# Autodesk Inventor assembly: 21.1846 LEVELING FOOT M10 WITH BORES
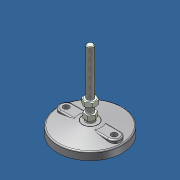
[picture p0: Inventor's stored thumbnail of the model, 180x180]
Saved by Autodesk Inventor 2016 (Build 200138000, 138)
## iProperties
Created: 2007-03-29
Part Number: 21.1846 LEVELING FOOT M10 WITH BORES
Document SubType Name: Assembly
Designer: Andy Moles
Author: Andy Moles
## Documents named in this file (5)
- C:\Users\myhome\Documents\Inventor\Printer\21.1846 LEVELING FOOT M10 WITH BORES.iam
- C:\Users\myhome\Documents\Inventor\Printer\LevelingFeet\ANTI-SKID PAD 100mm WITH BORES.ipt
- C:\Users\myhome\Documents\Inventor\Printer\LevelingFeet\PAD 100mm GRAY PLASTIC WITH BORES.IPT
- C:\Users\myhome\Documents\Inventor\Printer\LevelingFeet\21.1846 THREADED STUD 10mm.ipt
- C:\Users\myhome\Documents\Inventor\Printer\LevelingFeet\HEX NUT M10 DIN 934.ipt
## Components (4 placed, 4 different names)
1. ANTI-SKID PAD 100mm WITH BORES:1 — Insert:1, Mate:4
2. PAD 100mm GRAY PLASTIC WITH BORES:1 — Insert:1, Tangent:1, Mate:1, Mate:4
3. 21.1846 THREADED STUD 10mm:1 — Tangent:1, Mate:1, Mate:2
4. M10 HEX NUT DIN 934:1 — Mate:2
## Relationships (5: Mate 3, Insert 1, Tangent 1)
- Insert:1: ANTI-SKID PAD 100mm WITH BORES:1 ↔ PAD 100mm GRAY PLASTIC WITH BORES:1
- Tangent:1: PAD 100mm GRAY PLASTIC WITH BORES:1 ↔ 21.1846 THREADED STUD 10mm:1
- Mate:1: PAD 100mm GRAY PLASTIC WITH BORES:1 ↔ 21.1846 THREADED STUD 10mm:1
- Mate:2: 21.1846 THREADED STUD 10mm:1 ↔ M10 HEX NUT DIN 934:1
- Mate:4: ANTI-SKID PAD 100mm WITH BORES:1 ↔ PAD 100mm GRAY PLASTIC WITH BORES:1
